# Autodesk Inventor assembly: linear_cutting_endeffector-5
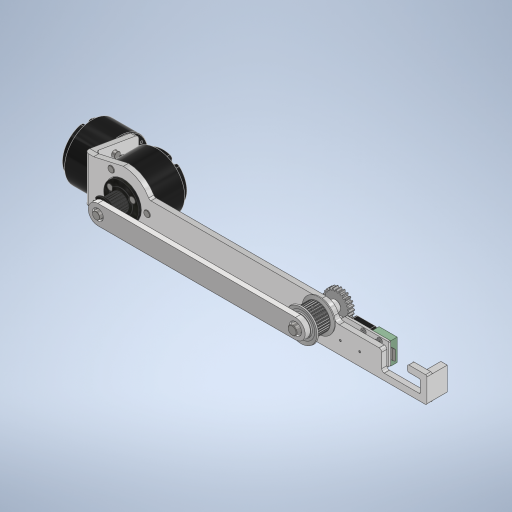
[picture p0: Inventor's stored thumbnail of the model, 512x512]
Saved by Autodesk Inventor 2024 (Build 280153000, 153)
## iProperties
Created: 2025-06-13
Part Number: linear_cutting_endeffector-5
Document SubType Name: Assembly
Designer: 1412z
Author: 1412z
## Documents named in this file (30)
- C:\Users\1412z\OneDrive\デスクトップ\rdclab\harvesting_robot\harvesting_endeffector\linear_cutting_endeffector\linear_cutting_endeffector-5.iam
- C:\Users\1412z\OneDrive\デスクトップ\rdclab\harvesting_robot\harvesting_endeffector\linear_cutting_endeffector\motor_holder\motor_holder-5.ipt
- C:\Users\1412z\OneDrive\デスクトップ\rdclab\harvesting_robot\harvesting_endeffector\linear_cutting_endeffector\misumi\SSE2B6L-100_Autodesk_Inventor_2023_20250607\AIS2023\SSE2B6-100_r.ipt
- C:\Users\1412z\OneDrive\デスクトップ\rdclab\harvesting_robot\harvesting_endeffector\linear_cutting_endeffector\misumi\screw\NBK_SNZSM26\SNZS-M2-6.ipt
- C:\Users\1412z\OneDrive\デスクトップ\rdclab\harvesting_robot\harvesting_endeffector\linear_cutting_endeffector\misumi\SSE2B6L-100_Autodesk_Inventor_2023_20250607\AIS2023\SSEB6_b.ipt
- C:\Users\1412z\OneDrive\デスクトップ\rdclab\harvesting_robot\harvesting_endeffector\linear_cutting_endeffector\misumi\meviy\slider_plate.ipt
- C:\Users\1412z\OneDrive\デスクトップ\rdclab\harvesting_robot\harvesting_endeffector\linear_cutting_endeffector\misumi\LRGEAM0.8KA-80-K2-B50_Autodesk_Inventor_2024_20250607\LRGEAM0_8KA-80-K2-B50.ipt
- C:\Users\1412z\OneDrive\デスクトップ\rdclab\harvesting_robot\harvesting_endeffector\linear_cutting_endeffector\misumi\pipe\Φ3.6-Φ2.2-4.ipt
- C:\Users\1412z\OneDrive\デスクトップ\rdclab\harvesting_robot\harvesting_endeffector\linear_cutting_endeffector\misumi\screw\CBSTSR2-3_Inventor\CBSTSR2-3.ipt
- C:\Users\1412z\OneDrive\デスクトップ\rdclab\harvesting_robot\harvesting_endeffector\linear_cutting_endeffector\misumi\screw\CBSTSR2-8_Inventor\CBSTSR2-8.ipt
- C:\Users\1412z\OneDrive\デスクトップ\rdclab\harvesting_robot\harvesting_endeffector\linear_cutting_endeffector\cutter\pen_type_cutter_realsize.ipt
- C:\Users\1412z\OneDrive\デスクトップ\rdclab\harvesting_robot\harvesting_endeffector\linear_cutting_endeffector\cutter\cutter_holder-2.ipt
- C:\Users\1412z\OneDrive\デスクトップ\rdclab\harvesting_robot\harvesting_endeffector\linear_cutting_endeffector\cutter\greiper_TPU.ipt
- C:\Users\1412z\OneDrive\デスクトップ\rdclab\harvesting_robot\harvesting_endeffector\linear_cutting_endeffector\GIM3505-08\GIM3505-8_with-driver.ipt
- C:\Users\1412z\OneDrive\デスクトップ\rdclab\harvesting_robot\harvesting_endeffector\linear_cutting_endeffector\misumi\C-FL675ZZ_Autodesk_Inventor_2024_20250608\C-FL675ZZ.ipt
- C:\Users\1412z\OneDrive\デスクトップ\rdclab\harvesting_robot\harvesting_endeffector\linear_cutting_endeffector\misumi\simring\simring_Φ5-Φ7.ipt
- C:\Users\1412z\OneDrive\デスクトップ\rdclab\harvesting_robot\harvesting_endeffector\linear_cutting_endeffector\misumi\HTPA32S2M100-A-P5_Autodesk_Inventor_2024_20250608\AIS2024\HTPA32S2M100-A-P5.iam
- C:\Users\1412z\OneDrive\デスクトップ\rdclab\harvesting_robot\harvesting_endeffector\linear_cutting_endeffector\misumi\HTPA22S2M100-A-V4-Z6-J3_Autodesk_Inventor_2024_20250304\HTPA22S2M100-A-V4-Z6-J3_0_a-3.ipt
- C:\Users\1412z\OneDrive\デスクトップ\rdclab\harvesting_robot\harvesting_endeffector\linear_cutting_endeffector\misumi\screw\M2.5×4\M2.5×4.ipt
- C:\Users\1412z\OneDrive\デスクトップ\rdclab\harvesting_robot\harvesting_endeffector\linear_cutting_endeffector\motor_holder\motor_holder_top-2.ipt
- C:\Users\1412z\OneDrive\デスクトップ\rdclab\harvesting_robot\harvesting_endeffector\linear_cutting_endeffector\misumi\SFL674ZZ_Autodesk_Inventor_2024_20250304\SFL674ZZ.ipt
- C:\Users\1412z\OneDrive\デスクトップ\rdclab\harvesting_robot\harvesting_endeffector\linear_cutting_endeffector\misumi\screw\M3×8\M3×8.ipt
- C:\Users\1412z\OneDrive\デスクトップ\rdclab\harvesting_robot\harvesting_endeffector\linear_cutting_endeffector\misumi\screw\M3×4\M3×4.ipt
- C:\Users\1412z\OneDrive\デスクトップ\rdclab\harvesting_robot\harvesting_endeffector\linear_cutting_endeffector\misumi\shaft\shaft_15.05.ipt
- C:\Users\1412z\OneDrive\デスクトップ\rdclab\harvesting_robot\harvesting_endeffector\linear_cutting_endeffector\misumi\washer\washer_M4.ipt
- C:\Users\1412z\OneDrive\デスクトップ\rdclab\harvesting_robot\harvesting_endeffector\linear_cutting_endeffector\misumi\shaft\shaft_34mm_Φ5.ipt
- C:\Users\1412z\OneDrive\デスクトップ\rdclab\harvesting_robot\harvesting_endeffector\linear_cutting_endeffector\misumi\screw\M4×5\M4×5.ipt
- C:\Users\1412z\OneDrive\デスクトップ\rdclab\harvesting_robot\harvesting_endeffector\linear_cutting_endeffector\misumi\CLBPS5-8-7_Autodesk_Inventor_2024_20250613\CLBPS5-8-7.ipt
- C:\Users\1412z\OneDrive\デスクトップ\rdclab\harvesting_robot\harvesting_endeffector\linear_cutting_endeffector\misumi\M0.8-24\Spur Gear (24 teeth).ipt
- C:\Users\1412z\OneDrive\デスクトップ\rdclab\harvesting_robot\harvesting_endeffector\linear_cutting_endeffector\misumi\MBIS2-3-4_Autodesk_Inventor_2023_20250613\AIS2023\MBIS2-3-4.ipt
## Components (56 placed, 29 different names)
1. motor_holder-5:1 — 回転:1, 回転:2, 回転:23, 回転:24, 回転:25, 回転:26, 回転:27, 回転:28, 回転:37, 回転:38, 回転:39, 回転:40, 回転:41, 回転:42
2. SSE2B6-100_r:1 — 回転:1, 回転:2, 回転:3, リジッド:1, 回転:4, 回転:5, 回転:6, 回転:7, 回転:8, 円柱状:1, 円柱状:2
3. SNZS-M2-6:1 — 回転:8
4. SNZS-M2-6:2 — 回転:7
5. SNZS-M2-6:3 — 回転:6
6. SNZS-M2-6:4 — 回転:5
7. SNZS-M2-6:5 — 回転:4
8. SNZS-M2-6:6 — リジッド:1
9. SNZS-M2-6:7 — 回転:3
10. SSEB6_b:1 — 円柱状:1, 回転:10
11. SSEB6_b:2 — 円柱状:2, 回転:9
12. slider_plate:1 — 回転:9, 回転:10, 回転:11, 回転:12, 回転:15, 回転:16, 回転:19, 回転:20, 回転:21, 回転:22, 回転:54, 回転:55, 回転:58, 回転:59
13. LRGEAM0_8KA-80-K2-B50:1 — 回転:11, 回転:12, 回転:13, 回転:14
14. Φ3.6-Φ2.2-4:1 — 回転:13, 回転:18
15. Φ3.6-Φ2.2-4:2 — 回転:14, 回転:17
16. CBSTSR2-3:1 — 回転:15
17. CBSTSR2-3:2 — 回転:16
18. CBSTSR2-8:1 — 回転:18
19. CBSTSR2-8:2 — 回転:17
20. pen_type_cutter_realsize:1 — リジッド:2
21. cutter_holder-2:1 — 回転:19, 回転:20, リジッド:2
22. greiper_TPU:1 — 回転:21, 回転:22, 回転:56, 回転:57
23. GIM3505-8_with-driver:1 — 回転:23, 回転:24, 回転:32, 回転:33
24. GIM3505-8_with-driver:2 — 回転:25, 回転:26
25. C-FL675ZZ:1 — 回転:27, 回転:29
26. C-FL675ZZ:2 — 回転:28, 回転:30
27. simring_Φ5-Φ7:1 — 回転:30, 回転:31
28. simring_Φ5-Φ7:2 — 回転:29, 回転:52
29. HTPA32S2M100-A-P5:1 [sub-assembly] — 回転:31, 回転:43
30. HTPA22S2M100-A-V4-Z6-J3_0_a-3:1 — 回転:32, 回転:33, 回転:34, 回転:35, 回転:36, 回転:44, 回転:47
31. M2.5×4:1 — 回転:36
32. M2.5×4:2 — 回転:38
33. M2.5×4:3 — 回転:34
34. M2.5×4:4 — 回転:37
35. M2.5×4:5 — 回転:35
36. M2.5×4:6 — 回転:39
37. M2.5×4:7 — 回転:42
38. M2.5×4:8 — 回転:40
39. M2.5×4:9 — 回転:41
40. motor_holder_top-2:1 — 回転:43, 回転:44, 回転:45, 回転:46
41. C-FL675ZZ:3 — 回転:45, 回転:50
42. SFL674ZZ:1 — 回転:46, 回転:48
43. M3×8:1 — リジッド:3
44. M3×4:1 — 回転:49
45. shaft_15.05:1 — 回転:48, 回転:49
46. washer_M4:1 — 回転:47, リジッド:3
47. shaft_34mm_Φ5:1 — 回転:50, 回転:51
48. M4×5:1 — 回転:51
49. CLBPS5-8-7:1 — 回転:52, 回転:53
50. Spur Gear (24 teeth):1 — 回転:53
51. CBSTSR2-3:3 — 回転:55
52. CBSTSR2-3:4 — 回転:54
53. MBIS2-3-4:1 — 回転:57
54. MBIS2-3-4:2 — 回転:56
55. CBSTSR2-3:5 — 回転:58
56. CBSTSR2-3:6 — 回転:59
## Relationships (64: RevoluteJoint 59, WeldJoint 3, CylindricalJoint 2)
- 回転:1 [RevoluteJoint]: motor_holder-5:1 ↔ SSE2B6-100_r:1
- 回転:2 [RevoluteJoint]: motor_holder-5:1 ↔ SSE2B6-100_r:1
- 回転:3 [RevoluteJoint]: SSE2B6-100_r:1 ↔ SNZS-M2-6:7
- リジッド:1 [WeldJoint]: SSE2B6-100_r:1 ↔ SNZS-M2-6:6
- 回転:4 [RevoluteJoint]: SSE2B6-100_r:1 ↔ SNZS-M2-6:5
- 回転:5 [RevoluteJoint]: SSE2B6-100_r:1 ↔ SNZS-M2-6:4
- 回転:6 [RevoluteJoint]: SSE2B6-100_r:1 ↔ SNZS-M2-6:3
- 回転:7 [RevoluteJoint]: SSE2B6-100_r:1 ↔ SNZS-M2-6:2
- 回転:8 [RevoluteJoint]: SSE2B6-100_r:1 ↔ SNZS-M2-6:1
- 円柱状:1 [CylindricalJoint]: SSE2B6-100_r:1 ↔ SSEB6_b:1
- 円柱状:2 [CylindricalJoint]: SSE2B6-100_r:1 ↔ SSEB6_b:2
- 回転:9 [RevoluteJoint]: SSEB6_b:2 ↔ slider_plate:1
- 回転:10 [RevoluteJoint]: SSEB6_b:1 ↔ slider_plate:1
- 回転:11 [RevoluteJoint]: slider_plate:1 ↔ LRGEAM0_8KA-80-K2-B50:1
- 回転:12 [RevoluteJoint]: slider_plate:1 ↔ LRGEAM0_8KA-80-K2-B50:1
- 回転:13 [RevoluteJoint]: LRGEAM0_8KA-80-K2-B50:1 ↔ Φ3.6-Φ2.2-4:1
- 回転:14 [RevoluteJoint]: LRGEAM0_8KA-80-K2-B50:1 ↔ Φ3.6-Φ2.2-4:2
- 回転:15 [RevoluteJoint]: slider_plate:1 ↔ CBSTSR2-3:1
- 回転:16 [RevoluteJoint]: slider_plate:1 ↔ CBSTSR2-3:2
- 回転:17 [RevoluteJoint]: Φ3.6-Φ2.2-4:2 ↔ CBSTSR2-8:2
- 回転:18 [RevoluteJoint]: Φ3.6-Φ2.2-4:1 ↔ CBSTSR2-8:1
- 回転:19 [RevoluteJoint]: slider_plate:1 ↔ cutter_holder-2:1
- 回転:20 [RevoluteJoint]: slider_plate:1 ↔ cutter_holder-2:1
- リジッド:2 [WeldJoint]: pen_type_cutter_realsize:1 ↔ cutter_holder-2:1
- 回転:21 [RevoluteJoint]: slider_plate:1 ↔ greiper_TPU:1
- 回転:22 [RevoluteJoint]: slider_plate:1 ↔ greiper_TPU:1
- 回転:23 [RevoluteJoint]: motor_holder-5:1 ↔ GIM3505-8_with-driver:1
- 回転:24 [RevoluteJoint]: motor_holder-5:1 ↔ GIM3505-8_with-driver:1
- 回転:25 [RevoluteJoint]: motor_holder-5:1 ↔ GIM3505-8_with-driver:2
- 回転:26 [RevoluteJoint]: motor_holder-5:1 ↔ GIM3505-8_with-driver:2
- 回転:27 [RevoluteJoint]: motor_holder-5:1 ↔ C-FL675ZZ:1
- 回転:28 [RevoluteJoint]: motor_holder-5:1 ↔ C-FL675ZZ:2
- 回転:29 [RevoluteJoint]: C-FL675ZZ:1 ↔ simring_Φ5-Φ7:2
- 回転:30 [RevoluteJoint]: C-FL675ZZ:2 ↔ simring_Φ5-Φ7:1
- 回転:31 [RevoluteJoint]: simring_Φ5-Φ7:1 ↔ HTPA32S2M100-A-P5:1
- 回転:32 [RevoluteJoint]: GIM3505-8_with-driver:1 ↔ HTPA22S2M100-A-V4-Z6-J3_0_a-3:1
- 回転:33 [RevoluteJoint]: GIM3505-8_with-driver:1 ↔ HTPA22S2M100-A-V4-Z6-J3_0_a-3:1
- 回転:34 [RevoluteJoint]: HTPA22S2M100-A-V4-Z6-J3_0_a-3:1 ↔ M2.5×4:3
- 回転:35 [RevoluteJoint]: HTPA22S2M100-A-V4-Z6-J3_0_a-3:1 ↔ M2.5×4:5
- 回転:36 [RevoluteJoint]: HTPA22S2M100-A-V4-Z6-J3_0_a-3:1 ↔ M2.5×4:1
- 回転:37 [RevoluteJoint]: motor_holder-5:1 ↔ M2.5×4:4
- 回転:38 [RevoluteJoint]: motor_holder-5:1 ↔ M2.5×4:2
- 回転:39 [RevoluteJoint]: motor_holder-5:1 ↔ M2.5×4:6
- 回転:40 [RevoluteJoint]: motor_holder-5:1 ↔ M2.5×4:8
- 回転:41 [RevoluteJoint]: motor_holder-5:1 ↔ M2.5×4:9
- 回転:42 [RevoluteJoint]: motor_holder-5:1 ↔ M2.5×4:7
- 回転:43 [RevoluteJoint]: HTPA32S2M100-A-P5:1 ↔ motor_holder_top-2:1
- 回転:44 [RevoluteJoint]: HTPA22S2M100-A-V4-Z6-J3_0_a-3:1 ↔ motor_holder_top-2:1
- 回転:45 [RevoluteJoint]: motor_holder_top-2:1 ↔ C-FL675ZZ:3
- 回転:46 [RevoluteJoint]: motor_holder_top-2:1 ↔ SFL674ZZ:1
- 回転:47 [RevoluteJoint]: HTPA22S2M100-A-V4-Z6-J3_0_a-3:1 ↔ washer_M4:1
- 回転:48 [RevoluteJoint]: SFL674ZZ:1 ↔ shaft_15.05:1
- リジッド:3 [WeldJoint]: M3×8:1 ↔ washer_M4:1
- 回転:49 [RevoluteJoint]: M3×4:1 ↔ shaft_15.05:1
- 回転:50 [RevoluteJoint]: C-FL675ZZ:3 ↔ shaft_34mm_Φ5:1
- 回転:51 [RevoluteJoint]: shaft_34mm_Φ5:1 ↔ M4×5:1
- 回転:52 [RevoluteJoint]: simring_Φ5-Φ7:2 ↔ CLBPS5-8-7:1
- 回転:53 [RevoluteJoint]: CLBPS5-8-7:1 ↔ Spur Gear (24 teeth):1
- 回転:54 [RevoluteJoint]: slider_plate:1 ↔ CBSTSR2-3:4
- 回転:55 [RevoluteJoint]: slider_plate:1 ↔ CBSTSR2-3:3
- 回転:56 [RevoluteJoint]: greiper_TPU:1 ↔ MBIS2-3-4:2
- 回転:57 [RevoluteJoint]: greiper_TPU:1 ↔ MBIS2-3-4:1
- 回転:58 [RevoluteJoint]: slider_plate:1 ↔ CBSTSR2-3:5
- 回転:59 [RevoluteJoint]: slider_plate:1 ↔ CBSTSR2-3:6
